# Autodesk Inventor assembly: Trabalho Final_999_001
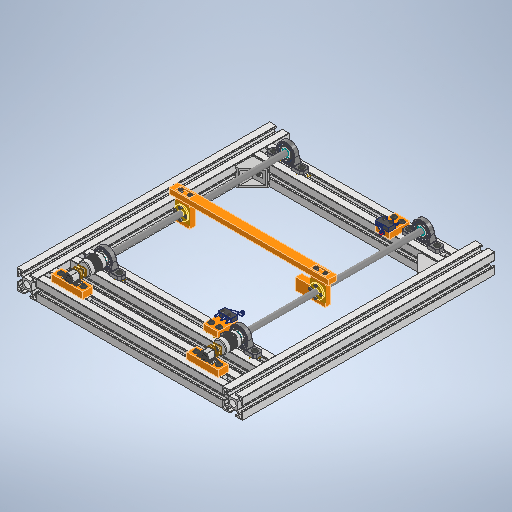
[picture p0: Inventor's stored thumbnail of the model, 512x512]
Saved by Autodesk Inventor 2026 (Build 300175000, 175)
## iProperties
Created: 2025-04-08
Part Number: Trabalho Final_999_001
Document SubType Name: Assembly
Designer: Carlos Dias
Author: Carlos Dias
## Documents named in this file (28)
- C:\Users\carlo\Documents\TEARCI-GIT\Projetos Pessoais\Eixo trapezoidal-Movimento Linear\Design\Inventor\Trabalho Final_999_001.iam
- C:\Users\carlo\Documents\TEARCI-GIT\Projetos Pessoais\Eixo trapezoidal-Movimento Linear\Design\Inventor\perfil_30x30_002.ipt
- C:\Users\carlo\Documents\TEARCI-GIT\Projetos Pessoais\Eixo trapezoidal-Movimento Linear\Design\Inventor\N10 DC Gear Motor\N10 DC Gear Motor\N10 DC Gear Motor.ipt
- C:\Users\carlo\Documents\TEARCI-GIT\Projetos Pessoais\Eixo trapezoidal-Movimento Linear\Design\Inventor\perfil_30x30_003.ipt
- C:\Users\carlo\Documents\TEARCI-GIT\Projetos Pessoais\Eixo trapezoidal-Movimento Linear\Design\Inventor\KP08 SUPPORT BEARING\KP08 SUPPORT BEARING\KP08 SUPPORT BEARING.ipt
- C:\Users\carlo\Documents\TEARCI-GIT\Projetos Pessoais\Eixo trapezoidal-Movimento Linear\Design\Inventor\6mmX9mmCoupler\6mmX9mmCoupler\6mmX9mmCoupler.ipt
- C:\Users\carlo\Documents\TEARCI-GIT\Projetos Pessoais\Eixo trapezoidal-Movimento Linear\Design\Inventor\porca_roscada_trapezoidal_001.ipt
- C:\Users\carlo\Documents\TEARCI-GIT\Projetos Pessoais\Eixo trapezoidal-Movimento Linear\Design\Inventor\eixo_trapesoidal_001.ipt
- C:\Users\carlo\Documents\TEARCI-GIT\Projetos Pessoais\Eixo trapezoidal-Movimento Linear\Design\Inventor\conector_motor_001.ipt
- C:\Users\carlo\Documents\Inventor\Content Center Files\R2026\en-US\ISO 4027\ISO 4027 - M2 x 8 - ISO.ipt
- C:\Users\carlo\Documents\TEARCI-GIT\Projetos Pessoais\Eixo trapezoidal-Movimento Linear\Design\Inventor\Microswitch\Microswitch\Microswitch.ipt
- C:\Users\carlo\Documents\TEARCI-GIT\Projetos Pessoais\Eixo trapezoidal-Movimento Linear\Design\Inventor\suporte_microswitch_001.ipt
- C:\Users\carlo\Documents\TEARCI-GIT\Projetos Pessoais\Eixo trapezoidal-Movimento Linear\Design\Inventor\batente_microswitch_001.ipt
- C:\Users\carlo\Documents\TEARCI-GIT\Projetos Pessoais\Eixo trapezoidal-Movimento Linear\Design\Inventor\suporte_motor_001.ipt
- C:\Users\carlo\Documents\TEARCI-GIT\Projetos Pessoais\Eixo trapezoidal-Movimento Linear\Design\Inventor\CBR3030\CBR3030\CBR3030.ipt
- C:\Users\carlo\Documents\Inventor\Content Center Files\R2026\en-US\ISO 7380-1\ISO 7380-1 - M4 x 10.ipt
- C:\Users\carlo\Documents\TEARCI-GIT\Projetos Pessoais\Eixo trapezoidal-Movimento Linear\Design\Inventor\BTN08M4\BTN08M4\BTN08M4.ipt
- C:\Users\carlo\Documents\Inventor\Content Center Files\R2026\en-US\ISO 7380-1\ISO 7380-1 - M4 x 12.ipt
- C:\Users\carlo\Documents\TEARCI-GIT\Projetos Pessoais\Eixo trapezoidal-Movimento Linear\Design\Inventor\BPN08M4\BPN08M4\BPN08M4.ipt
- C:\Users\carlo\Documents\Inventor\Content Center Files\R2026\en-US\ISO 7380-1\ISO 7380-1 - M4 x 16.ipt
- C:\Users\carlo\Documents\Inventor\Content Center Files\R2026\en-US\ISO 4762(2)\ISO 4762 - M2 x 12ISO.ipt
- C:\Users\carlo\Documents\TEARCI-GIT\Projetos Pessoais\Eixo trapezoidal-Movimento Linear\Design\Inventor\rosca_trapezoidal_001.ipt
- C:\Users\carlo\Documents\TEARCI-GIT\Projetos Pessoais\Eixo trapezoidal-Movimento Linear\Design\Inventor\conector_eixos_001.ipt
- C:\Users\carlo\Documents\Inventor\Content Center Files\R2026\en-US\ISO 4762(2)\ISO 4762 - M3 x 12ISO.ipt
- C:\Users\carlo\Documents\Inventor\Content Center Files\R2026\en-US\ISO 4762(2)\ISO 4762 - M2 x 8ISO.ipt
- C:\Users\carlo\Documents\Inventor\Content Center Files\R2026\en-US\ISO 4027\ISO 4027 - M1,6 x 2 - ISO.ipt
- C:\Users\carlo\Documents\TEARCI-GIT\Projetos Pessoais\Eixo trapezoidal-Movimento Linear\Design\Inventor\chapa_motor_001.ipt
- C:\Users\carlo\Documents\Inventor\Content Center Files\R2026\en-US\ISO 4762(2)\ISO 4762 - M2 x 5ISO.ipt
## Components (112 placed, 27 different names)
1. perfil_30x30_002:1 — Mate:1, Mate:2, Flush:1, Mate:5, Mate:6, Flush:2, Mate:12, Mate:13, Mate:147, Mate:247, Mate:250, Mate:251
2. perfil_30x30_003:2 — Mate:7, Mate:8, Flush:5, Mate:29, Flush:8, Mate:42, Flush:70, Mate:100, Mate:128, Flush:73, Mate:132, Mate:134, Flush:77, Flush:83, Mate:161, Mate:237, Mate:244, Mate:245, Mate:246, Mate:248, Mate:282, Flush:92, Mate:283, Mate:284
3. perfil_30x30_002:2 — Mate:12, Mate:13, Flush:5, Mate:29, Mate:92, Flush:75, Mate:137, Mate:138
4. perfil_30x30_003:3 — Mate:9, Mate:10, Mate:11, Mate:23, Flush:64, Mate:63, Mate:67, Mate:68, Mate:71, Mate:79, Mate:157, Mate:158
5. perfil_30x30_003:1 — Mate:5, Mate:6, Flush:2, Mate:7, Mate:8, Mate:9, Mate:10, Mate:11, Mate:51, Mate:52, Mate:89, Mate:94, Flush:79, Flush:80, Mate:141, Mate:142, Mate:143, Mate:144
6. CBR3030:2 — Mate:244, Mate:246, Mate:249, Flush:87, Mate:251, Mate:253, Mate:255
7. BPN08M4:9 — Mate:245, Mate:248, Mate:249, Mate:252
8. ISO 7380-1 M4 x 16:13 — Mate:254, Mate:255
9. BPN08M4:10 — Mate:247, Mate:250, Flush:87, Mate:254
10. ISO 7380-1 M4 x 16:14 — Mate:252, Mate:253
11. conector_eixos_001:1 — Mate:197, Mate:200, Mate:202, Mate:203, Mate:212, Mate:213, Mate:214, Mate:215, Mate:216, Mate:217, Mate:218, Mate:219
12. BPN08M4:5 — Flush:75, Mate:132, Flush:76, Mate:133
13. ISO 7380-1 M4 x 16:5 — Mate:133, Mate:135
14. BPN08M4:6 — Flush:78, Mate:137, Mate:140
15. ISO 7380-1 M4 x 16:6 — Mate:139
16. CBR3030:1 — Flush:76, Mate:134, Mate:135, Flush:77, Mate:138, Mate:139, Mate:140
17. ISO 4762 M2 x 12:2 — Mate:108, Mate:109
18. ISO 4762 M2 x 12:1 — Mate:110, Mate:111
19. Microswitch:1 — Mate:43, Mate:44, Mate:45, Mate:108, Mate:109, Mate:110, Mate:111
20. suporte_microswitch_001:1 — Mate:43, Mate:44, Mate:45, Mate:69, Mate:70, Mate:71, Mate:73, Mate:74, Mate:76, Mate:77, Mate:107
21. BTN08M4:2 — Flush:65, Mate:67, Flush:66, Mate:70, Mate:75
22. BTN08M4:3 — Flush:66, Mate:68, Mate:69, Mate:72, Flush:67
23. ISO 7380-1 M4 x 12:1 — Mate:75, Mate:76, Mate:77
24. ISO 7380-1 M4 x 12:2 — Mate:72, Mate:73, Mate:74
25. Microswitch:3 — Mate:236, Mate:238, Mate:239, Mate:240, Mate:241, Mate:242, Mate:243
26. suporte_microswitch_001:2 — Mate:131, Mate:236, Mate:237, Mate:238, Mate:239
27. BTN08M4:5 — Mate:128, Flush:73, Flush:74, Mate:129
28. BTN08M4:6 — Flush:74, Mate:130
29. ISO 7380-1 M4 x 12:3 — Mate:130
30. ISO 7380-1 M4 x 12:4 — Mate:129
31. ISO 4762 M2 x 12:3 — Mate:240, Mate:243
32. ISO 4762 M2 x 12:4 — Mate:241, Mate:242
33. ISO 4762 M2 x 5:5 — Mate:275, Mate:278
34. ISO 4762 M2 x 5:6 — Mate:277, Mate:281
35. ISO 4762 M2 x 5:7 — Mate:274, Mate:279
36. ISO 4762 M2 x 5:8 — Mate:276, Mate:280
37. ISO 4027 M1,6 x 2:7 — Mate:262, Tangent:7
38. ISO 4027 M1,6 x 2:8 — Mate:263, Tangent:8
39. chapa_motor_001:1 — Flush:88, Mate:264, Flush:89, Mate:278, Mate:279, Mate:280, Mate:281
40. ISO 4027 M1,6 x 2:2 — Mate:256, Tangent:1
41. ISO 4027 M1,6 x 2:1 — Mate:257, Tangent:2
42. ISO 4762 M2 x 8:6 — Mate:222, Mate:227
43. ISO 4762 M3 x 12:1 — Mate:213, Mate:215
44. ISO 4762 M3 x 12:2 — Mate:212, Mate:214
45. batente_microswitch_001:1 — Mate:194, Mate:198, Mate:201, Mate:202
46. porca_roscada_trapezoidal_001:1 — Mate:193, Mate:198, Mate:201, Mate:220, Mate:221, Mate:222, Mate:223, Mate:224, Mate:225, Mate:226, Mate:227
47. N10 DC Gear Motor:1 — Mate:31, Mate:32, Mate:38, Mate:54, Flush:10, Flush:11, Mate:264, Flush:89
48. KP08 SUPPORT BEARING:2 — Mate:23, Mate:30, Mate:65, Mate:66, Mate:80, Mate:81, Mate:82, Mate:107, Mate:112, Mate:256, Mate:257
49. 6mmX9mmCoupler:1 — Mate:33, Mate:34, Mate:36, Mate:38, Mate:40, Mate:59, Mate:60, Mate:112
50. eixo_trapesoidal_001:1 — Mate:30, Mate:40, Mate:41, Flush:9, Mate:61, Mate:62, Mate:193, Mate:194, Tangent:1, Tangent:2, Tangent:7, Tangent:8
51. ISO 4762 M3 x 12:3 — Mate:216, Mate:218
52. ISO 4762 M3 x 12:4 — Mate:217, Mate:219
53. ISO 4762 M2 x 8:1 — Mate:220, Mate:221
54. ISO 4762 M2 x 8:2 — Mate:223, Mate:226
55. ISO 4762 M2 x 8:3 — Mate:224, Mate:225
56. conector_motor_001:1 — Mate:31, Mate:32, Mate:33, Mate:35, Mate:37
57. ISO 4027 M2 x 8:2 — Mate:34, Mate:35
58. ISO 4027 M2 x 8:3 — Mate:36, Mate:37
59. KP08 SUPPORT BEARING:3 — Mate:41, Flush:8, Mate:42, Flush:9, Mate:101, Mate:102, Mate:103, Mate:104, Mate:105, Mate:106, Mate:131, Mate:262, Mate:263
60. suporte_motor_001:1 — Mate:51, Mate:52, Mate:54, Flush:10, Flush:11, Mate:92, Mate:93, Mate:95, Mate:96, Mate:97, Mate:98, Mate:99, Flush:88, Mate:274, Mate:275, Mate:276, Mate:277
61. ISO 4027 M2 x 8:4 — Mate:59, Mate:62
62. ISO 4027 M2 x 8:5 — Mate:60, Mate:61
63. BTN08M4:1 — Flush:64, Mate:63, Mate:64, Flush:65
64. ISO 7380-1 M4 x 10:1 — Mate:64, Mate:65, Mate:66
65. BTN08M4:4 — Flush:67, Mate:79, Mate:80
66. ISO 7380-1 M4 x 10:2 — Mate:81, Mate:82
67. BPN08M4:1 — Mate:89, Mate:93, Flush:68
68. BPN08M4:2 — Flush:68, Mate:94, Mate:95
69. ISO 7380-1 M4 x 16:1 — Mate:96, Mate:98
70. ISO 7380-1 M4 x 16:2 — Mate:97, Mate:99
71. BPN08M4:3 — Flush:70, Flush:71, Mate:100, Mate:102
72. BPN08M4:4 — Flush:71, Mate:101
73. ISO 7380-1 M4 x 16:3 — Mate:103, Mate:104
74. ISO 7380-1 M4 x 16:4 — Mate:105, Mate:106
75. BPN08M4:11 — Flush:92, Mate:283, Mate:286
76. BPN08M4:12 — Mate:282, Mate:284, Mate:285
77. chapa_motor_001:2 — Flush:90, Flush:91, Mate:265, Mate:270, Mate:271, Mate:272, Mate:273
78. ISO 4762 M2 x 5:1 — Mate:266, Mate:271
79. ISO 4762 M2 x 5:2 — Mate:267, Mate:270
80. ISO 4762 M2 x 5:3 — Mate:268, Mate:273
81. ISO 4762 M2 x 5:4 — Mate:269, Mate:272
82. ISO 4027 M1,6 x 2:3 — Mate:258, Tangent:3
83. ISO 4027 M1,6 x 2:4 — Mate:259, Tangent:4
84. ISO 4027 M1,6 x 2:5 — Mate:260, Tangent:5
85. ISO 4027 M1,6 x 2:6 — Mate:261, Tangent:6
86. ISO 4762 M2 x 8:8 — Mate:229, Mate:233
87. ISO 4762 M2 x 8:7 — Mate:230, Mate:232
88. ISO 4762 M2 x 8:4 — Mate:228, Mate:235
89. ISO 4762 M2 x 8:5 — Mate:231, Mate:234
90. porca_roscada_trapezoidal_001:2 — Mate:192, Mate:196, Mate:199, Mate:228, Mate:229, Mate:230, Mate:231, Mate:232, Mate:233, Mate:234, Mate:235
91. rosca_trapezoidal_001:1 — Mate:195, Mate:196, Mate:197, Mate:199, Mate:200, Mate:203
92. ISO 7380-1 M4 x 16:12 — Mate:188, Mate:191, Mate:285
93. ISO 7380-1 M4 x 16:11 — Mate:189, Mate:190, Mate:286
94. ISO 7380-1 M4 x 16:7 — Mate:183, Mate:185
95. ISO 7380-1 M4 x 16:8 — Mate:182, Mate:184
96. ISO 7380-1 M4 x 16:9 — Mate:181, Mate:187
97. ISO 7380-1 M4 x 16:10 — Mate:180, Mate:186
98. ISO 4027 M2 x 8:6 — Mate:172, Mate:173
99. ISO 4027 M2 x 8:7 — Mate:174, Mate:175
100. ISO 4027 M2 x 8:8 — Mate:176, Mate:178
101. ISO 4027 M2 x 8:9 — Mate:177, Mate:179
102. KP08 SUPPORT BEARING:5 — Flush:83, Mate:161, Mate:162, Flush:84, Mate:188, Mate:189, Mate:190, Mate:191, Mate:260, Mate:261
103. N10 DC Gear Motor:2 — Mate:155, Mate:156, Mate:265
104. KP08 SUPPORT BEARING:4 — Mate:157, Mate:159, Mate:160, Mate:180, Mate:181, Mate:186, Mate:187, Mate:258, Mate:259
105. 6mmX9mmCoupler:2 — Mate:172, Mate:174, Mate:176, Mate:177
106. eixo_trapesoidal_001:2 — Mate:162, Flush:84, Mate:178, Mate:179, Mate:192, Mate:195, Tangent:3, Tangent:4, Tangent:5, Tangent:6
107. conector_motor_001:2 — Mate:173, Mate:175
108. BTN08M4:7 — Flush:81, Flush:82, Mate:158, Mate:159
109. BTN08M4:8 — Flush:81, Flush:82, Mate:160
110. BPN08M4:7 — Flush:80, Mate:141, Mate:146
111. BPN08M4:8 — Flush:79, Mate:142, Mate:145
112. suporte_motor_001:2 — Mate:143, Mate:144, Mate:145, Mate:146, Mate:147, Mate:155, Mate:156, Mate:182, Mate:183, Mate:184, Mate:185, Flush:90, Flush:91, Mate:266, Mate:267, Mate:268, Mate:269
## Relationships (265: Mate 223, Flush 34, Tangent 8)
- Mate:1: perfil_30x30_002:1
- Mate:2: perfil_30x30_002:1
- Flush:1: perfil_30x30_002:1
- Mate:5: perfil_30x30_002:1 ↔ perfil_30x30_003:1
- Mate:6: perfil_30x30_002:1 ↔ perfil_30x30_003:1
- Flush:2: perfil_30x30_002:1 ↔ perfil_30x30_003:1
- Mate:7: perfil_30x30_003:2 ↔ perfil_30x30_003:1
- Mate:8: perfil_30x30_003:2 ↔ perfil_30x30_003:1
- Mate:9: perfil_30x30_003:3 ↔ perfil_30x30_003:1
- Mate:10: perfil_30x30_003:3 ↔ perfil_30x30_003:1
- Mate:11 (-80 mm): perfil_30x30_003:3 ↔ perfil_30x30_003:1
- Mate:12: perfil_30x30_002:1 ↔ perfil_30x30_002:2
- Mate:13: perfil_30x30_002:1 ↔ perfil_30x30_002:2
- Mate:23: perfil_30x30_003:3 ↔ KP08 SUPPORT BEARING:2
- Flush:5 (25 mm): perfil_30x30_003:2 ↔ perfil_30x30_002:2
- Mate:29: perfil_30x30_003:2 ↔ perfil_30x30_002:2
- Mate:30: KP08 SUPPORT BEARING:2 ↔ eixo_trapesoidal_001:1
- Mate:31: N10 DC Gear Motor:1 ↔ conector_motor_001:1
- Mate:32: N10 DC Gear Motor:1 ↔ conector_motor_001:1
- Mate:33: 6mmX9mmCoupler:1 ↔ conector_motor_001:1
- Mate:34: 6mmX9mmCoupler:1 ↔ ISO 4027 M2 x 8:2
- Mate:35: conector_motor_001:1 ↔ ISO 4027 M2 x 8:2
- Mate:36: 6mmX9mmCoupler:1 ↔ ISO 4027 M2 x 8:3
- Mate:37: conector_motor_001:1 ↔ ISO 4027 M2 x 8:3
- Mate:38 (3 mm): N10 DC Gear Motor:1 ↔ 6mmX9mmCoupler:1
- Mate:40: 6mmX9mmCoupler:1 ↔ eixo_trapesoidal_001:1
- Mate:41: eixo_trapesoidal_001:1 ↔ KP08 SUPPORT BEARING:3
- Flush:8: perfil_30x30_003:2 ↔ KP08 SUPPORT BEARING:3
- Mate:42: perfil_30x30_003:2 ↔ KP08 SUPPORT BEARING:3
- Flush:9 (-2.5 mm): eixo_trapesoidal_001:1 ↔ KP08 SUPPORT BEARING:3
- Mate:43: Microswitch:1 ↔ suporte_microswitch_001:1
- Mate:44: Microswitch:1 ↔ suporte_microswitch_001:1
- Mate:45: Microswitch:1 ↔ suporte_microswitch_001:1
- Mate:51: perfil_30x30_003:1 ↔ suporte_motor_001:1
- Mate:52: perfil_30x30_003:1 ↔ suporte_motor_001:1
- Mate:54: N10 DC Gear Motor:1 ↔ suporte_motor_001:1
- Flush:10: N10 DC Gear Motor:1 ↔ suporte_motor_001:1
- Flush:11 (1.5 mm): N10 DC Gear Motor:1 ↔ suporte_motor_001:1
- Mate:59: 6mmX9mmCoupler:1 ↔ ISO 4027 M2 x 8:4
- Mate:60: 6mmX9mmCoupler:1 ↔ ISO 4027 M2 x 8:5
- Mate:61: eixo_trapesoidal_001:1 ↔ ISO 4027 M2 x 8:5
- Mate:62: eixo_trapesoidal_001:1 ↔ ISO 4027 M2 x 8:4
- Flush:64: perfil_30x30_003:3 ↔ BTN08M4:1
- Mate:63 (0.4 mm): perfil_30x30_003:3 ↔ BTN08M4:1
- Mate:64: BTN08M4:1 ↔ ISO 7380-1 M4 x 10:1
- Mate:65: KP08 SUPPORT BEARING:2 ↔ ISO 7380-1 M4 x 10:1
- Mate:66: KP08 SUPPORT BEARING:2 ↔ ISO 7380-1 M4 x 10:1
- Flush:65: BTN08M4:2 ↔ BTN08M4:1
- Mate:67 (0.4 mm): perfil_30x30_003:3 ↔ BTN08M4:2
- Flush:66: BTN08M4:2 ↔ BTN08M4:3
- Mate:68 (0.4 mm): perfil_30x30_003:3 ↔ BTN08M4:3
- Mate:69: suporte_microswitch_001:1 ↔ BTN08M4:3
- Mate:70: suporte_microswitch_001:1 ↔ BTN08M4:2
- Mate:71: perfil_30x30_003:3 ↔ suporte_microswitch_001:1
- Mate:72: BTN08M4:3 ↔ ISO 7380-1 M4 x 12:2
- Mate:73: suporte_microswitch_001:1 ↔ ISO 7380-1 M4 x 12:2
- Mate:74: suporte_microswitch_001:1 ↔ ISO 7380-1 M4 x 12:2
- Mate:75: BTN08M4:2 ↔ ISO 7380-1 M4 x 12:1
- Mate:76: suporte_microswitch_001:1 ↔ ISO 7380-1 M4 x 12:1
- Mate:77: suporte_microswitch_001:1 ↔ ISO 7380-1 M4 x 12:1
- [Mate]: BTN08M4:4 ↔ ISO 7380-1 M4 x 10:2
- Flush:67: BTN08M4:3 ↔ BTN08M4:4
- Mate:79: perfil_30x30_003:3 ↔ BTN08M4:4
- Mate:80: KP08 SUPPORT BEARING:2 ↔ BTN08M4:4
- Mate:81: KP08 SUPPORT BEARING:2 ↔ ISO 7380-1 M4 x 10:2
- Mate:82: KP08 SUPPORT BEARING:2 ↔ ISO 7380-1 M4 x 10:2
- Mate:89: perfil_30x30_003:1 ↔ BPN08M4:1
- Mate:92 (15 mm): perfil_30x30_002:2 ↔ suporte_motor_001:1
- Mate:93: suporte_motor_001:1 ↔ BPN08M4:1
- Flush:68: BPN08M4:1 ↔ BPN08M4:2
- Mate:94: perfil_30x30_003:1 ↔ BPN08M4:2
- Mate:95: suporte_motor_001:1 ↔ BPN08M4:2
- Mate:96: suporte_motor_001:1 ↔ ISO 7380-1 M4 x 16:1
- Mate:97: suporte_motor_001:1 ↔ ISO 7380-1 M4 x 16:2
- Mate:98: suporte_motor_001:1 ↔ ISO 7380-1 M4 x 16:1
- Mate:99: suporte_motor_001:1 ↔ ISO 7380-1 M4 x 16:2
- [Flush]: BPN08M4:3 ↔ BPN08M4:4
- Flush:70: perfil_30x30_003:2 ↔ BPN08M4:3
- Flush:71: BPN08M4:3 ↔ BPN08M4:4
- Mate:100: perfil_30x30_003:2 ↔ BPN08M4:3
- Mate:101: KP08 SUPPORT BEARING:3 ↔ BPN08M4:4
- Mate:102: KP08 SUPPORT BEARING:3 ↔ BPN08M4:3
- Mate:103: KP08 SUPPORT BEARING:3 ↔ ISO 7380-1 M4 x 16:3
- Mate:104: KP08 SUPPORT BEARING:3 ↔ ISO 7380-1 M4 x 16:3
- Mate:105: KP08 SUPPORT BEARING:3 ↔ ISO 7380-1 M4 x 16:4
- Mate:106: KP08 SUPPORT BEARING:3 ↔ ISO 7380-1 M4 x 16:4
- Mate:107: suporte_microswitch_001:1 ↔ KP08 SUPPORT BEARING:2
- Mate:108: ISO 4762 M2 x 12:2 ↔ Microswitch:1
- Mate:109: ISO 4762 M2 x 12:2 ↔ Microswitch:1
- Mate:110: ISO 4762 M2 x 12:1 ↔ Microswitch:1
- Mate:111: ISO 4762 M2 x 12:1 ↔ Microswitch:1
- Mate:112 (2 mm): KP08 SUPPORT BEARING:2 ↔ 6mmX9mmCoupler:1
- [Flush]: BTN08M4:5 ↔ BTN08M4:6
- [Mate]: suporte_microswitch_001:2 ↔ ISO 7380-1 M4 x 12:4
- [Mate]: suporte_microswitch_001:2 ↔ ISO 7380-1 M4 x 12:4
- [Mate]: suporte_microswitch_001:2 ↔ ISO 7380-1 M4 x 12:3
- [Mate]: suporte_microswitch_001:2 ↔ ISO 7380-1 M4 x 12:3
- Mate:128 (0.4 mm): perfil_30x30_003:2 ↔ BTN08M4:5
- Flush:73: perfil_30x30_003:2 ↔ BTN08M4:5
- Flush:74: BTN08M4:5 ↔ BTN08M4:6
- Mate:129: BTN08M4:5 ↔ ISO 7380-1 M4 x 12:4
- Mate:130: BTN08M4:6 ↔ ISO 7380-1 M4 x 12:3
- Mate:131: suporte_microswitch_001:2 ↔ KP08 SUPPORT BEARING:3
- Flush:75: perfil_30x30_002:2 ↔ BPN08M4:5
- Mate:132: perfil_30x30_003:2 ↔ BPN08M4:5
- Flush:76: BPN08M4:5 ↔ CBR3030:1
- Mate:133: BPN08M4:5 ↔ ISO 7380-1 M4 x 16:5
- Mate:134: perfil_30x30_003:2 ↔ CBR3030:1
- Mate:135: ISO 7380-1 M4 x 16:5 ↔ CBR3030:1
- Flush:77: perfil_30x30_003:2 ↔ CBR3030:1
- [Mate]: BPN08M4:6 ↔ ISO 7380-1 M4 x 16:6
- Flush:78: BPN08M4:6
- Mate:137: perfil_30x30_002:2 ↔ BPN08M4:6
- Mate:138: perfil_30x30_002:2 ↔ CBR3030:1
- Mate:139: ISO 7380-1 M4 x 16:6 ↔ CBR3030:1
- Mate:140: BPN08M4:6 ↔ CBR3030:1
- Flush:79: perfil_30x30_003:1 ↔ BPN08M4:8
- Flush:80: perfil_30x30_003:1 ↔ BPN08M4:7
- Mate:141: perfil_30x30_003:1 ↔ BPN08M4:7
- Mate:142: perfil_30x30_003:1 ↔ BPN08M4:8
- Mate:143: perfil_30x30_003:1 ↔ suporte_motor_001:2
- Mate:144: perfil_30x30_003:1 ↔ suporte_motor_001:2
- Mate:145: BPN08M4:8 ↔ suporte_motor_001:2
- Mate:146: BPN08M4:7 ↔ suporte_motor_001:2
- Mate:147 (15 mm): perfil_30x30_002:1 ↔ suporte_motor_001:2
- [Mate]: KP08 SUPPORT BEARING:4 ↔ eixo_trapesoidal_001:2
- [Mate]: N10 DC Gear Motor:2 ↔ conector_motor_001:2
- [Mate]: N10 DC Gear Motor:2 ↔ conector_motor_001:2
- [Mate]: 6mmX9mmCoupler:2 ↔ conector_motor_001:2
- [Mate] (3 mm): N10 DC Gear Motor:2 ↔ 6mmX9mmCoupler:2
- [Mate]: 6mmX9mmCoupler:2 ↔ eixo_trapesoidal_001:2
- [Mate] (2 mm): KP08 SUPPORT BEARING:4 ↔ 6mmX9mmCoupler:2
- Mate:155: N10 DC Gear Motor:2 ↔ suporte_motor_001:2
- Mate:156: N10 DC Gear Motor:2 ↔ suporte_motor_001:2
- Mate:157: perfil_30x30_003:3 ↔ KP08 SUPPORT BEARING:4
- Flush:81: BTN08M4:7 ↔ BTN08M4:8
- Flush:82: BTN08M4:7 ↔ BTN08M4:8
- Mate:158 (0.4 mm): perfil_30x30_003:3 ↔ BTN08M4:7
- Mate:159: KP08 SUPPORT BEARING:4 ↔ BTN08M4:7
- Mate:160: KP08 SUPPORT BEARING:4 ↔ BTN08M4:8
- Flush:83: perfil_30x30_003:2 ↔ KP08 SUPPORT BEARING:5
- Mate:161: perfil_30x30_003:2 ↔ KP08 SUPPORT BEARING:5
- Mate:162: KP08 SUPPORT BEARING:5 ↔ eixo_trapesoidal_001:2
- Flush:84 (-2.5 mm): KP08 SUPPORT BEARING:5 ↔ eixo_trapesoidal_001:2
- Mate:172: ISO 4027 M2 x 8:6 ↔ 6mmX9mmCoupler:2
- Mate:173: ISO 4027 M2 x 8:6 ↔ conector_motor_001:2
- Mate:174: ISO 4027 M2 x 8:7 ↔ 6mmX9mmCoupler:2
- Mate:175: ISO 4027 M2 x 8:7 ↔ conector_motor_001:2
- Mate:176: ISO 4027 M2 x 8:8 ↔ 6mmX9mmCoupler:2
- Mate:177: ISO 4027 M2 x 8:9 ↔ 6mmX9mmCoupler:2
- Mate:178: ISO 4027 M2 x 8:8 ↔ eixo_trapesoidal_001:2
- Mate:179: ISO 4027 M2 x 8:9 ↔ eixo_trapesoidal_001:2
- Mate:180: ISO 7380-1 M4 x 16:10 ↔ KP08 SUPPORT BEARING:4
- Mate:181: ISO 7380-1 M4 x 16:9 ↔ KP08 SUPPORT BEARING:4
- Mate:182: ISO 7380-1 M4 x 16:8 ↔ suporte_motor_001:2
- Mate:183: ISO 7380-1 M4 x 16:7 ↔ suporte_motor_001:2
- Mate:184: ISO 7380-1 M4 x 16:8 ↔ suporte_motor_001:2
- Mate:185: ISO 7380-1 M4 x 16:7 ↔ suporte_motor_001:2
- Mate:186: ISO 7380-1 M4 x 16:10 ↔ KP08 SUPPORT BEARING:4
- Mate:187: ISO 7380-1 M4 x 16:9 ↔ KP08 SUPPORT BEARING:4
- Mate:188: ISO 7380-1 M4 x 16:12 ↔ KP08 SUPPORT BEARING:5
- Mate:189: ISO 7380-1 M4 x 16:11 ↔ KP08 SUPPORT BEARING:5
- Mate:190: ISO 7380-1 M4 x 16:11 ↔ KP08 SUPPORT BEARING:5
- Mate:191: ISO 7380-1 M4 x 16:12 ↔ KP08 SUPPORT BEARING:5
- Mate:192: porca_roscada_trapezoidal_001:2 ↔ eixo_trapesoidal_001:2
- Mate:193: porca_roscada_trapezoidal_001:1 ↔ eixo_trapesoidal_001:1
- Mate:194: batente_microswitch_001:1 ↔ eixo_trapesoidal_001:1
- Mate:195: rosca_trapezoidal_001:1 ↔ eixo_trapesoidal_001:2
- Mate:196: porca_roscada_trapezoidal_001:2 ↔ rosca_trapezoidal_001:1
- Mate:197: conector_eixos_001:1 ↔ rosca_trapezoidal_001:1
- Mate:198: batente_microswitch_001:1 ↔ porca_roscada_trapezoidal_001:1
- Mate:199: porca_roscada_trapezoidal_001:2 ↔ rosca_trapezoidal_001:1
- Mate:200: conector_eixos_001:1 ↔ rosca_trapezoidal_001:1
- Mate:201: batente_microswitch_001:1 ↔ porca_roscada_trapezoidal_001:1
- Mate:202: conector_eixos_001:1 ↔ batente_microswitch_001:1
- Mate:203: conector_eixos_001:1 ↔ rosca_trapezoidal_001:1
- Mate:212: conector_eixos_001:1 ↔ ISO 4762 M3 x 12:2
- Mate:213: conector_eixos_001:1 ↔ ISO 4762 M3 x 12:1
- Mate:214: conector_eixos_001:1 ↔ ISO 4762 M3 x 12:2
- Mate:215: conector_eixos_001:1 ↔ ISO 4762 M3 x 12:1
- Mate:216: conector_eixos_001:1 ↔ ISO 4762 M3 x 12:3
- Mate:217: conector_eixos_001:1 ↔ ISO 4762 M3 x 12:4
- Mate:218: conector_eixos_001:1 ↔ ISO 4762 M3 x 12:3
- Mate:219: conector_eixos_001:1 ↔ ISO 4762 M3 x 12:4
- Mate:220: porca_roscada_trapezoidal_001:1 ↔ ISO 4762 M2 x 8:1
- Mate:221: porca_roscada_trapezoidal_001:1 ↔ ISO 4762 M2 x 8:1
- Mate:222: ISO 4762 M2 x 8:6 ↔ porca_roscada_trapezoidal_001:1
- Mate:223: porca_roscada_trapezoidal_001:1 ↔ ISO 4762 M2 x 8:2
- Mate:224: porca_roscada_trapezoidal_001:1 ↔ ISO 4762 M2 x 8:3
- Mate:225: porca_roscada_trapezoidal_001:1 ↔ ISO 4762 M2 x 8:3
- Mate:226: porca_roscada_trapezoidal_001:1 ↔ ISO 4762 M2 x 8:2
- Mate:227: ISO 4762 M2 x 8:6 ↔ porca_roscada_trapezoidal_001:1
- Mate:228: ISO 4762 M2 x 8:4 ↔ porca_roscada_trapezoidal_001:2
- Mate:229: ISO 4762 M2 x 8:8 ↔ porca_roscada_trapezoidal_001:2
- Mate:230: ISO 4762 M2 x 8:7 ↔ porca_roscada_trapezoidal_001:2
- Mate:231: ISO 4762 M2 x 8:5 ↔ porca_roscada_trapezoidal_001:2
- Mate:232: ISO 4762 M2 x 8:7 ↔ porca_roscada_trapezoidal_001:2
- Mate:233: ISO 4762 M2 x 8:8 ↔ porca_roscada_trapezoidal_001:2
- Mate:234: ISO 4762 M2 x 8:5 ↔ porca_roscada_trapezoidal_001:2
- Mate:235: ISO 4762 M2 x 8:4 ↔ porca_roscada_trapezoidal_001:2
- Mate:236: Microswitch:3 ↔ suporte_microswitch_001:2
- Mate:237: perfil_30x30_003:2 ↔ suporte_microswitch_001:2
- Mate:238: Microswitch:3 ↔ suporte_microswitch_001:2
- Mate:239: Microswitch:3 ↔ suporte_microswitch_001:2
- Mate:240: Microswitch:3 ↔ ISO 4762 M2 x 12:3
- Mate:241: Microswitch:3 ↔ ISO 4762 M2 x 12:4
- Mate:242: Microswitch:3 ↔ ISO 4762 M2 x 12:4
- Mate:243: Microswitch:3 ↔ ISO 4762 M2 x 12:3
- Mate:244: perfil_30x30_003:2 ↔ CBR3030:2
- Mate:245: perfil_30x30_003:2 ↔ BPN08M4:9
- Mate:246: perfil_30x30_003:2 ↔ CBR3030:2
- Mate:247: perfil_30x30_002:1 ↔ BPN08M4:10
- Mate:248: perfil_30x30_003:2 ↔ BPN08M4:9
- Mate:249: CBR3030:2 ↔ BPN08M4:9
- Mate:250: perfil_30x30_002:1 ↔ BPN08M4:10
- Flush:87: CBR3030:2 ↔ BPN08M4:10
- Mate:251: perfil_30x30_002:1 ↔ CBR3030:2
- Mate:252: BPN08M4:9 ↔ ISO 7380-1 M4 x 16:14
- Mate:253: CBR3030:2 ↔ ISO 7380-1 M4 x 16:14
- Mate:254: ISO 7380-1 M4 x 16:13 ↔ BPN08M4:10
- Mate:255: CBR3030:2 ↔ ISO 7380-1 M4 x 16:13
- Mate:256: ISO 4027 M1,6 x 2:2 ↔ KP08 SUPPORT BEARING:2
- Tangent:1: ISO 4027 M1,6 x 2:2 ↔ eixo_trapesoidal_001:1
- Mate:257: ISO 4027 M1,6 x 2:1 ↔ KP08 SUPPORT BEARING:2
- Tangent:2: ISO 4027 M1,6 x 2:1 ↔ eixo_trapesoidal_001:1
- Mate:258: ISO 4027 M1,6 x 2:3 ↔ KP08 SUPPORT BEARING:4
- Mate:259: ISO 4027 M1,6 x 2:4 ↔ KP08 SUPPORT BEARING:4
- Tangent:3: ISO 4027 M1,6 x 2:3 ↔ eixo_trapesoidal_001:2
- Tangent:4: ISO 4027 M1,6 x 2:4 ↔ eixo_trapesoidal_001:2
- Mate:260: ISO 4027 M1,6 x 2:5 ↔ KP08 SUPPORT BEARING:5
- Tangent:5: ISO 4027 M1,6 x 2:5 ↔ eixo_trapesoidal_001:2
- Mate:261: ISO 4027 M1,6 x 2:6 ↔ KP08 SUPPORT BEARING:5
- Tangent:6: ISO 4027 M1,6 x 2:6 ↔ eixo_trapesoidal_001:2
- Mate:262: ISO 4027 M1,6 x 2:7 ↔ KP08 SUPPORT BEARING:3
- Mate:263: ISO 4027 M1,6 x 2:8 ↔ KP08 SUPPORT BEARING:3
- Tangent:7: ISO 4027 M1,6 x 2:7 ↔ eixo_trapesoidal_001:1
- Tangent:8: ISO 4027 M1,6 x 2:8 ↔ eixo_trapesoidal_001:1
- Flush:88: chapa_motor_001:1 ↔ suporte_motor_001:1
- Mate:264: chapa_motor_001:1 ↔ N10 DC Gear Motor:1
- Flush:89: chapa_motor_001:1 ↔ N10 DC Gear Motor:1
- Flush:90: chapa_motor_001:2 ↔ suporte_motor_001:2
- Flush:91: chapa_motor_001:2 ↔ suporte_motor_001:2
- Mate:265: chapa_motor_001:2 ↔ N10 DC Gear Motor:2
- Mate:266: ISO 4762 M2 x 5:1 ↔ suporte_motor_001:2
- Mate:267: ISO 4762 M2 x 5:2 ↔ suporte_motor_001:2
- Mate:268: ISO 4762 M2 x 5:3 ↔ suporte_motor_001:2
- Mate:269: ISO 4762 M2 x 5:4 ↔ suporte_motor_001:2
- Mate:270: chapa_motor_001:2 ↔ ISO 4762 M2 x 5:2
- Mate:271: chapa_motor_001:2 ↔ ISO 4762 M2 x 5:1
- Mate:272: chapa_motor_001:2 ↔ ISO 4762 M2 x 5:4
- Mate:273: chapa_motor_001:2 ↔ ISO 4762 M2 x 5:3
- Mate:274: ISO 4762 M2 x 5:7 ↔ suporte_motor_001:1
- Mate:275: ISO 4762 M2 x 5:5 ↔ suporte_motor_001:1
- Mate:276: ISO 4762 M2 x 5:8 ↔ suporte_motor_001:1
- Mate:277: ISO 4762 M2 x 5:6 ↔ suporte_motor_001:1
- Mate:278: ISO 4762 M2 x 5:5 ↔ chapa_motor_001:1
- Mate:279: ISO 4762 M2 x 5:7 ↔ chapa_motor_001:1
- Mate:280: ISO 4762 M2 x 5:8 ↔ chapa_motor_001:1
- Mate:281: ISO 4762 M2 x 5:6 ↔ chapa_motor_001:1
- Mate:282: perfil_30x30_003:2 ↔ BPN08M4:12
- Flush:92: perfil_30x30_003:2 ↔ BPN08M4:11
- Mate:283: perfil_30x30_003:2 ↔ BPN08M4:11
- Mate:284: perfil_30x30_003:2 ↔ BPN08M4:12
- Mate:285: BPN08M4:12 ↔ ISO 7380-1 M4 x 16:12
- Mate:286: BPN08M4:11 ↔ ISO 7380-1 M4 x 16:11
## Named parameters: d172_d154 = 0 mm, d202_d191 = 0 mm, d219_d161 = 0 mm, d223_d167 = 0 mm, d224_d168 = 0 mm, d226_d170 = 0 mm, d227_d171 = 0 mm, d248_d244 = 0 mm, d317_d218 = 2 mm, d318_d89 = 0 mm, d319_d90 = 0 mm, d320_d91 = 0 mm, d321_d104 = 3 mm, d322_d108 = 0 mm, d323_d84 = 0 mm
